# Autodesk Inventor assembly: Claw Assembly
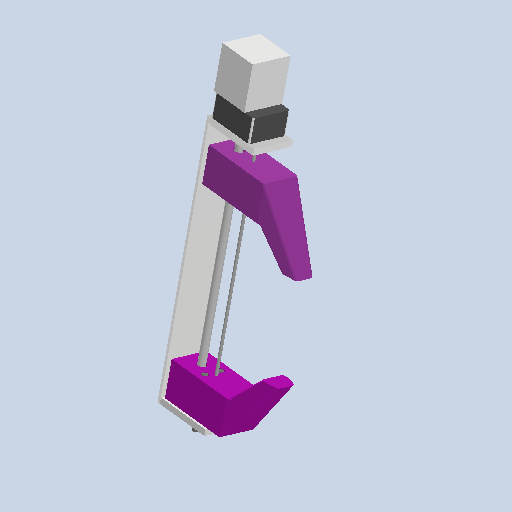
[picture p0: Inventor's stored thumbnail of the model, 512x512]
Saved by Autodesk Inventor 2025.1 (Build 291241020, 241B)
## iProperties
Created: 2025-01-21
Part Number: Claw Assembly
Document SubType Name: Assembly
Designer: Sven
Author: Sven
## Documents named in this file (12)
- C:\Users\t205b\OneDrive\Documents\Github\BehrendURCMechanical\CAD\Arm\Hamburger\BRC Robotic CLaw\Claw Assembly.iam
- C:\Users\t205b\OneDrive\Documents\Github\BehrendURCMechanical\CAD\Arm\Hamburger\BRC Robotic CLaw\Moving Gripper.ipt
- C:\Users\t205b\OneDrive\Documents\Github\BehrendURCMechanical\CAD\Arm\Hamburger\BRC Robotic CLaw\Stationary Gripper.ipt
- C:\Users\t205b\OneDrive\Documents\Github\BehrendURCMechanical\CAD\Arm\Hamburger\BRC Robotic CLaw\Lead Screw.ipt
- C:\Users\t205b\OneDrive\Documents\Github\BehrendURCMechanical\CAD\Arm\Hamburger\BRC Robotic CLaw\#10 2in.ipt
- C:\Users\t205b\OneDrive\Documents\Github\BehrendURCMechanical\CAD\Arm\Hamburger\BRC Robotic CLaw\Support Bar.ipt
- C:\Users\t205b\OneDrive\Documents\Github\BehrendURCMechanical\CAD\Arm\Hamburger\BRC Robotic CLaw\Motor Brace.ipt
- C:\Users\t205b\OneDrive\Documents\Github\BehrendURCMechanical\CAD\Arm\Hamburger\BRC Robotic CLaw\Couple.ipt
- C:\Users\t205b\OneDrive\Documents\Github\BehrendURCMechanical\CAD\Arm\Hamburger\BRC Robotic CLaw\NEMA 17 Completely Correct.ipt
- C:\Users\t205b\OneDrive\Documents\Github\BehrendURCMechanical\CAD\Arm\Hamburger\BRC Robotic CLaw\Bracket(left).ipt
- C:\Users\t205b\OneDrive\Documents\Github\BehrendURCMechanical\CAD\Arm\Hamburger\BRC Robotic CLaw\AR-BracketRight2.ipt
- C:\Users\t205b\OneDrive\Documents\Github\BehrendURCMechanical\CAD\Arm\Hamburger\BRC Robotic CLaw\AR-BracketMiddle2.ipt
## Components (12 placed, 11 different names)
1. Moving Gripper:1 — Mate:6, Mate:14, Mate:19, Mate:26
2. Stationary Gripper:1 — Mate:7, Mate:8, Mate:9, Mate:10, Mate:11, Mate:14, Mate:27, Mate:37
3. Lead Screw:1 — Mate:6, Mate:7, Mate:20, Mate:21, Mate:25, Mate:35, Mate:38
4. #10 2in:1 — Mate:8, Mate:9
5. #10 2in:2 — Mate:10, Mate:11
6. Support Bar:1 — Mate:26, Mate:27, Mate:33, Mate:39, Flush:1
7. Motor Brace:1 — Mate:19, Mate:30, Mate:31, Mate:32, Mate:33, Mate:34, Mate:36
8. Couple:1 — Mate:20, Mate:21, Mate:24, Mate:30
9. NEMA 17 Completely Correct:1 — Mate:24, Mate:25, Mate:31, Mate:32
10. AR-BracketRight2:1 — Mate:37, Mate:38, Mate:39, Flush:1, Mate:40, Mate:41, Mate:42
11. AR-BracketMiddle2:1 — Mate:40, Mate:41, Mate:42, Mate:43, Mate:44
12. Bracket(left):1 — Mate:34, Mate:35, Mate:36, Mate:43, Mate:44
## Relationships (30: Mate 29, Flush 1)
- Mate:6: Moving Gripper:1 ↔ Lead Screw:1
- Mate:7: Stationary Gripper:1 ↔ Lead Screw:1
- Mate:8: Stationary Gripper:1 ↔ #10 2in:1
- Mate:9: Stationary Gripper:1 ↔ #10 2in:1
- Mate:10: Stationary Gripper:1 ↔ #10 2in:2
- Mate:11: Stationary Gripper:1 ↔ #10 2in:2
- Mate:14: Moving Gripper:1 ↔ Stationary Gripper:1
- Mate:19: Moving Gripper:1 ↔ Motor Brace:1
- Mate:20: Lead Screw:1 ↔ Couple:1
- Mate:21: Lead Screw:1 ↔ Couple:1
- Mate:24: Couple:1 ↔ NEMA 17 Completely Correct:1
- Mate:25: Lead Screw:1 ↔ NEMA 17 Completely Correct:1
- Mate:26: Moving Gripper:1 ↔ Support Bar:1
- Mate:27: Stationary Gripper:1 ↔ Support Bar:1
- Mate:30: Motor Brace:1 ↔ Couple:1
- Mate:31: Motor Brace:1 ↔ NEMA 17 Completely Correct:1
- Mate:32: Motor Brace:1 ↔ NEMA 17 Completely Correct:1
- Mate:33: Support Bar:1 ↔ Motor Brace:1
- Mate:34: Motor Brace:1 ↔ Bracket(left):1
- Mate:35: Lead Screw:1 ↔ Bracket(left):1
- Mate:36: Motor Brace:1 ↔ Bracket(left):1
- Mate:37: Stationary Gripper:1 ↔ AR-BracketRight2:1
- Mate:38: Lead Screw:1 ↔ AR-BracketRight2:1
- Mate:39: Support Bar:1 ↔ AR-BracketRight2:1
- Flush:1: Support Bar:1 ↔ AR-BracketRight2:1
- Mate:40: AR-BracketRight2:1 ↔ AR-BracketMiddle2:1
- Mate:41: AR-BracketRight2:1 ↔ AR-BracketMiddle2:1
- Mate:42: AR-BracketRight2:1 ↔ AR-BracketMiddle2:1
- Mate:43: AR-BracketMiddle2:1 ↔ Bracket(left):1
- Mate:44: AR-BracketMiddle2:1 ↔ Bracket(left):1
